# Autodesk Inventor assembly: Hybrid
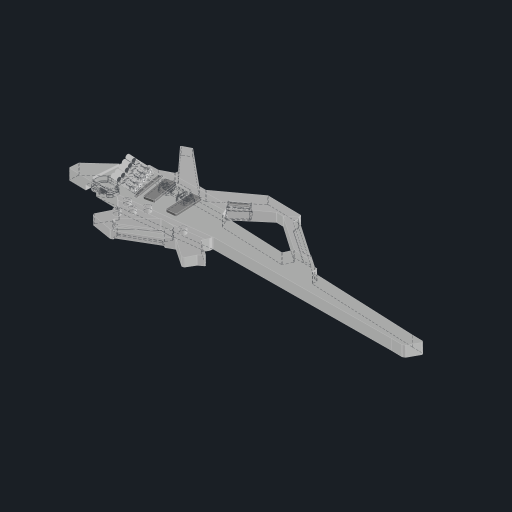
[picture p0: Inventor's stored thumbnail of the model, 512x512]
Saved by Autodesk Inventor 2023 (Build 270158000, 158)
## iProperties
Created: 2022-11-10
Part Number: Hybrid
Document SubType Name: Assembly
Designer: valer
Author: valer
## Documents named in this file (8)
- C:\Users\valer\Desktop\hybrid\src\Hybrid.iam
- C:\Users\valer\Desktop\hybrid\src\Hybrid.ipt
- C:\Users\valer\Desktop\hybrid\src\OscilloscopeScreen.ipt
- C:\Users\valer\Desktop\hybrid\src\BassTuner.ipt
- C:\Users\valer\Desktop\hybrid\src\MidiPickup.ipt
- C:\Users\valer\Desktop\hybrid\src\dpdt-switch-example.ipt
- C:\Users\valer\Desktop\hybrid\src\Panel.ipt
- C:\Users\valer\Desktop\hybrid\src\MidiController.ipt
## Components (12 placed, 7 different names)
1. Hybrid:1 — Flush:2, Mate:2, Mate:3, Mate:13, Mate:14, Mate:15, Mate:22, Flush:5, Mate:24, Mate:25
2. OscilloscopeScreen:1 — Flush:2, Mate:2, Mate:3
3. BassTuner:1
4. BassTuner:2
5. BassTuner:3
6. BassTuner:4
7. BassTuner:5
8. MidiPickup:1 — Mate:13
9. dpdt-switch-example:1 — Flush:3, Flush:4, Mate:20, Mate:23
10. dpdt-switch-example:2 — Flush:3, Flush:4, Mate:18, Mate:19
11. Panel:1 — Mate:14, Mate:15, Mate:18, Mate:19, Mate:20, Mate:22, Mate:23
12. MidiController:1 — Flush:5, Mate:24, Mate:25
## Relationships (16: Mate 12, Flush 4)
- Flush:2: Hybrid:1 ↔ OscilloscopeScreen:1
- Mate:2: Hybrid:1 ↔ OscilloscopeScreen:1
- Mate:3: Hybrid:1 ↔ OscilloscopeScreen:1
- Mate:13: Hybrid:1 ↔ MidiPickup:1
- Flush:3: dpdt-switch-example:1 ↔ dpdt-switch-example:2
- Flush:4: dpdt-switch-example:1 ↔ dpdt-switch-example:2
- Mate:14: Hybrid:1 ↔ Panel:1
- Mate:15: Hybrid:1 ↔ Panel:1
- Mate:18: dpdt-switch-example:2 ↔ Panel:1
- Mate:19: dpdt-switch-example:2 ↔ Panel:1
- Mate:20: dpdt-switch-example:1 ↔ Panel:1
- Mate:22: Hybrid:1 ↔ Panel:1
- Mate:23: dpdt-switch-example:1 ↔ Panel:1
- Flush:5 (-10 mm): Hybrid:1 ↔ MidiController:1
- Mate:24 (-152.4 mm): Hybrid:1 ↔ MidiController:1
- Mate:25: Hybrid:1 ↔ MidiController:1
